# Autodesk Inventor assembly: 8B
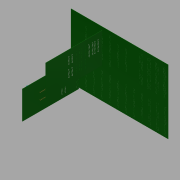
[picture p0: Inventor's stored thumbnail of the model, 180x180]
Saved by Autodesk Inventor 2019.4 (Build 234330000, 330)
## iProperties
Created: 2021-10-02
Part Number: 8B
Document SubType Name: Assembly
Designer: erics
Mass: 37.5522 g
Surface Area: 1305.02 cm^2
Volume: 37.5522 cm^3
Density: 1 g/cm^3
Author: erics
## Documents named in this file (4)
- D:\Users\erics\Documents\16B\Mechanical\8B.iam
- D:\Users\erics\Documents\16B\Backplane\Backplane.iam
- D:\Users\erics\Documents\16B\Memory_EEPROM\Memory_EEPROM_TOP.iam
- D:\Users\erics\Documents\16B\Program_Counter\Program_Counter.iam
## Components (3 placed, 3 different names)
1. Backplane:1 [sub-assembly] — Mate:1, Mate:2
2. Memory_EEPROM_TOP:1 [sub-assembly] — Mate:1
3. Program_Counter:1 [sub-assembly] — Mate:2
## Relationships (2: Mate 2)
- Mate:1 (2.54 mm): Backplane:1 ↔ Memory_EEPROM_TOP:1
- Mate:2 (2.54 mm): Backplane:1 ↔ Program_Counter:1
## Named parameters: CardToBP = 2.54 mm
